# Autodesk Inventor assembly: 1x11
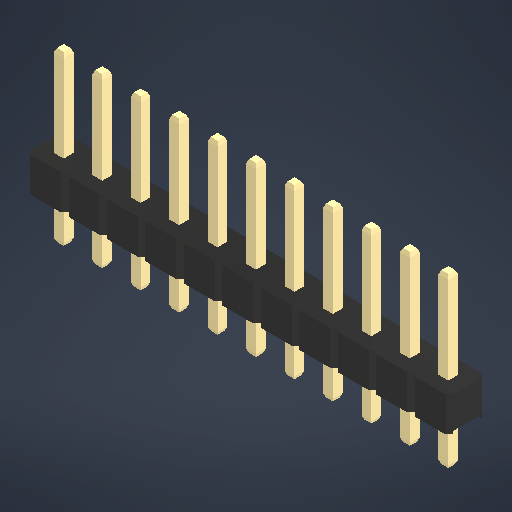
[picture p0: Inventor's stored thumbnail of the model, 512x512]
Saved by Autodesk Inventor 2026.1 (Build 301233020, 233B)
## iProperties
Created: 2020-05-13
Part Number: 1x11
Document SubType Name: Assembly
Designer: celio
Part Number: Assem_For_Pattern
Sending System: SOLIDWORKS 2018
Last Saved Date: 2020-05-13
last saved by: Vahagn
Author: celio
## Documents named in this file (2)
- C:\Users\celio\OneDrive\Documentos\Inventor\ZeGuia\Pinos\Macho\1x11\1x11.iam
- C:\Users\celio\OneDrive\Documentos\Inventor\Seguidor\Versão 1\Partes\male-pin-2-54-mm-1.snapshot.47\Assem_For_Pattern\Assem_For_Pattern\1_Male_Pin_2.54_mm.ipt
## Components (11 placed, 11 different names)
1. 1_Male_Pin_2.54_mm-1
2. 1_Male_Pin_2.54_mm-2
3. 1_Male_Pin_2.54_mm-3
4. 1_Male_Pin_2.54_mm-4
5. 1_Male_Pin_2.54_mm-5
6. 1_Male_Pin_2.54_mm-6
7. 1_Male_Pin_2.54_mm-7
8. 1_Male_Pin_2.54_mm-8
9. 1_Male_Pin_2.54_mm-9
10. 1_Male_Pin_2.54_mm-10 — Coincidente:1, Alinhado:1, Alinhado:2
11. 1_Male_Pin_2.54_mm:11 — Coincidente:1, Alinhado:1, Alinhado:2
## Relationships (3: Flush 2, Mate 1)
- Coincidente:1 [Mate]: 1_Male_Pin_2.54_mm-10 ↔ 1_Male_Pin_2.54_mm:11
- Alinhado:1 [Flush]: 1_Male_Pin_2.54_mm-10 ↔ 1_Male_Pin_2.54_mm:11
- Alinhado:2 [Flush]: 1_Male_Pin_2.54_mm-10 ↔ 1_Male_Pin_2.54_mm:11
